# Autodesk Inventor assembly: Feuerzeug
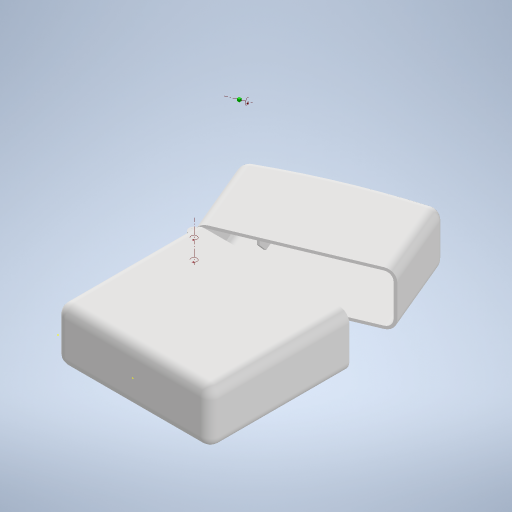
[picture p0: Inventor's stored thumbnail of the model, 512x512]
Saved by Autodesk Inventor 2023.2 (Build 272271000, 271)
## iProperties
Created: 2022-12-04
Part Number: Feuerzeug
Document SubType Name: Assembly
Designer: Koffermann
Author: Koffermann
## Documents named in this file (6)
- C:\Users\Koffermann\Documents\Funken Design\3D\Feuerzeug.iam
- C:\Users\Koffermann\Documents\Funken Design\3D\unteres_teil.ipt
- C:\Users\Koffermann\Documents\Funken Design\3D\oberes_teil.ipt
- C:\Users\Koffermann\Documents\Funken Design\3D\stab.ipt
- C:\Users\Koffermann\Documents\Funken Design\3D\verbindung_oben.ipt
- C:\Users\Koffermann\Documents\Funken Design\3D\verbindung_unten.ipt
## Components (5 placed, 5 different names)
1. unteres_teil:1 — Fluchtend:1, Fluchtend:2, Fluchtend:3, Passend:4, Passend:5, Passend:6, Drehung/Translation:1, Passend:11
2. oberes_teil:1 — Passend:1, Passend:2, Passend:3, Drehung/Translation:1
3. stab:1 — Passend:7, Passend:8, Passend:9, Passend:10, Passend:11
4. verbindung_oben:1 — Passend:1, Passend:2, Passend:3, Passend:7, Passend:8, Passend:9
5. verbindung_unten:1 — Passend:4, Passend:5, Passend:6, Passend:10
## Relationships (15: Mate 11, Flush 3, RelateRotateTranslate 1)
- Fluchtend:1 [Flush]: unteres_teil:1
- Fluchtend:2 [Flush]: unteres_teil:1
- Fluchtend:3 [Flush]: unteres_teil:1
- Passend:1 [Mate]: oberes_teil:1 ↔ verbindung_oben:1
- Passend:2 [Mate]: oberes_teil:1 ↔ verbindung_oben:1
- Passend:3 [Mate]: oberes_teil:1 ↔ verbindung_oben:1
- Passend:4 [Mate]: unteres_teil:1 ↔ verbindung_unten:1
- Passend:5 [Mate]: unteres_teil:1 ↔ verbindung_unten:1
- Passend:6 [Mate]: unteres_teil:1 ↔ verbindung_unten:1
- Passend:7 [Mate]: stab:1 ↔ verbindung_oben:1
- Passend:8 [Mate]: stab:1 ↔ verbindung_oben:1
- Passend:9 [Mate]: stab:1 ↔ verbindung_oben:1
- Drehung/Translation:1 [RelateRotateTranslate] (1 mm): unteres_teil:1 ↔ oberes_teil:1
- Passend:10 [Mate]: stab:1 ↔ verbindung_unten:1
- Passend:11 [Mate]: unteres_teil:1 ↔ stab:1
